# Autodesk Inventor assembly: BatPack
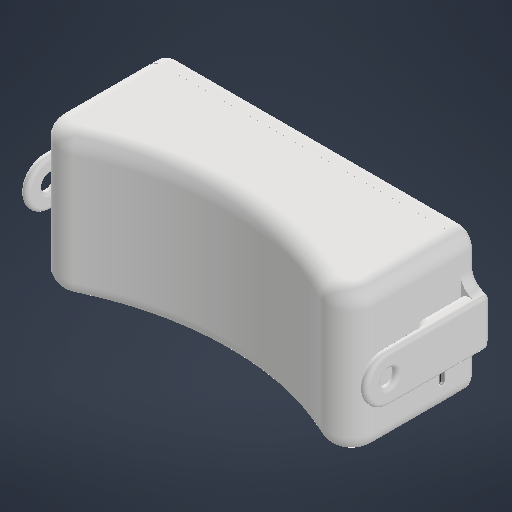
[picture p0: Inventor's stored thumbnail of the model, 512x512]
Saved by Autodesk Inventor 2025 (Build 290162000, 162)
## iProperties
Created: 2024-05-30
Part Number: BatPack
Document SubType Name: Assembly
Designer: techn
Author: techn
## Documents named in this file (5)
- C:\Users\techn\OneDrive\devMaxTrauma\3DModel\BatPack.iam
- C:\Users\techn\OneDrive\devMaxTrauma\3DModel\BatPackCase.ipt
- C:\Users\techn\OneDrive\devMaxTrauma\3DModel\xiaomi.ipt
- C:\Users\techn\OneDrive\devMaxTrauma\3DModel\usb-c-female-jrc-b008-1.snapshot.5\USB-C board JRC-B023\USB-C board JRC-B023.iam
- C:\Users\techn\OneDrive\devMaxTrauma\3DModel\BatPackCaseCover.ipt
## Components (5 placed, 4 different names)
1. BatPackCase:1 — Rigid:1, Rigid:3, Rigid:4
2. xiaomi:1 — Rigid:1, Rigid:2
3. xiaomi:2 — Rigid:2
4. USB-C board JRC-B023:1 [sub-assembly] — Rigid:3
5. BatPackCaseCover:1 — Rigid:4
## Relationships (4: WeldJoint 4)
- Rigid:1 [WeldJoint]: BatPackCase:1 ↔ xiaomi:1
- Rigid:2 [WeldJoint]: xiaomi:1 ↔ xiaomi:2
- Rigid:3 [WeldJoint]: BatPackCase:1 ↔ USB-C board JRC-B023:1
- Rigid:4 [WeldJoint]: BatPackCase:1 ↔ BatPackCaseCover:1
